# Autodesk Inventor assembly: Speaker
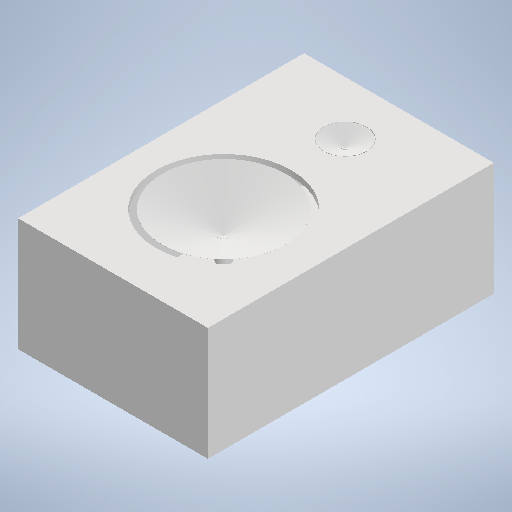
[picture p0: Inventor's stored thumbnail of the model, 512x512]
Saved by Autodesk Inventor 2025.2 (Build 292293000, 293)
## iProperties
Created: 2025-02-21
Part Number: Speaker
Document SubType Name: Assembly
Designer: fiste
Author: fiste
## Documents named in this file (7)
- C:\Users\fiste\Desktop\PhysikLautsprecher\Speaker.iam
- C:\Users\fiste\Desktop\PhysikLautsprecher\box_under.ipt
- C:\Users\fiste\Desktop\PhysikLautsprecher\membrane.ipt
- C:\Users\fiste\Desktop\PhysikLautsprecher\box_cover.ipt
- C:\Users\fiste\Desktop\PhysikLautsprecher\small_membrane.ipt
- C:\Users\fiste\Desktop\PhysikLautsprecher\small_membrane_shell.ipt
- C:\Users\fiste\Desktop\PhysikLautsprecher\small_membran_magnet.ipt
## Components (6 placed, 6 different names)
1. box_under:1 — Mate:1, Mate:2
2. membrane:1 — Rotational:1
3. box_cover:1 — Mate:1, Mate:2, Rotational:1, Rotational:2, Rotational:3
4. small_membrane:1 — Rotational:2
5. small_membrane_shell:1 — Rotational:3, Rigid:1
6. small_membran_magnet:1 — Rigid:1
## Relationships (6: RevoluteJoint 3, Mate 2, WeldJoint 1)
- Mate:1: box_under:1 ↔ box_cover:1
- Mate:2: box_under:1 ↔ box_cover:1
- Rotational:1 [RevoluteJoint]: membrane:1 ↔ box_cover:1
- Rotational:2 [RevoluteJoint]: box_cover:1 ↔ small_membrane:1
- Rotational:3 [RevoluteJoint]: box_cover:1 ↔ small_membrane_shell:1
- Rigid:1 [WeldJoint]: small_membrane_shell:1 ↔ small_membran_magnet:1
